# Autodesk Inventor assembly: Shooter Assembly
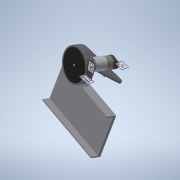
[picture p0: Inventor's stored thumbnail of the model, 180x180]
Saved by Autodesk Inventor 2021 (Build 250183000, 183)
## iProperties
Created: 2020-10-17
Part Number: Shooter Assembly
Document SubType Name: Assembly
Designer: Delta
Author: Delta
## Documents named in this file (12)
- D:\robotics\CAD\2020-21-CAD\Shooter\Shooter Assembly.iam
- D:\robotics\CAD\2020-21-CAD\Shooter\Guide.ipt
- D:\robotics\CAD\2020-21-CAD\Shooter\Axle Rotate.ipt
- D:\robotics\CAD\2020-21-CAD\Shooter\Triangle axle slide connector.ipt
- D:\robotics\CAD\2020-21-CAD\Shooter\Tetrex 2pc motor mount.ipt
- D:\robotics\CAD\2020-21-CAD\Shooter\motor-3102NeveRest20 (1).ipt
- D:\robotics\CAD\2020-21-CAD\Shooter\Flywheel_4inWheel8mmHub.ipt
- D:\robotics\CAD\2020-21-CAD\Shooter\Tetrix bracket - single servo.ipt
- D:\robotics\CAD\COTSParts\Rev\REV-41-1097SmartServo.ipt
- D:\robotics\CAD\2020-21-CAD\Shooter\Triangle connector.ipt
- D:\robotics\CAD\2020-21-CAD\Shooter\U bracket.ipt
- D:\robotics\CAD\2020-21-CAD\Shooter\Triangle connector 2.ipt
## Components (14 placed, 11 different names)
1. Guide:1 — Mate:14, Mate:15, Angle:1, Angle:2, Mate:37, Mate:38, Mate:39, Mate:40
2. Axle Rotate:1 — Mate:9, Mate:13, Mate:40
3. Axle Rotate:2 — Mate:8, Mate:12, Mate:37, Mate:38, Mate:39
4. Triangle axle slide connector:1 — Mate:8, Flush:2, Mate:12, Angle:3, Mate:34, Flush:5, Mate:35, Flush:7
5. Triangle axle slide connector:2 — Mate:9, Flush:2, Mate:13, Mate:24, Flush:3, Mate:30, Mate:31
6. Tetrex 2pc motor mount:1 — Mate:14, Mate:15, Angle:1, Mate:16, Mate:17
7. motor-3102NeveRest20 (1):1 — Mate:16, Mate:17, Mate:18, Mate:19, Angle:2
8. Flywheel_4inWheel8mmHub:1 — Mate:18, Mate:19
9. Tetrix bracket - single servo:1 — Mate:25, Mate:26, Mate:27, Angle:3, Mate:32, Flush:4
10. REV-41-1097SmartServo:1 — Mate:25, Mate:26, Mate:27, Mate:30
11. Triangle connector:1 — Mate:24, Flush:3, Mate:33, Flush:6
12. U bracket:1 — Mate:31, Mate:32, Flush:4, Mate:33
13. Triangle connector:2 — Mate:34, Flush:5, Flush:6, Mate:36
14. Triangle connector 2:1 — Mate:35, Flush:7, Mate:36
## Relationships (34: Mate 25, Flush 6, Angle 3)
- Mate:8: Axle Rotate:2 ↔ Triangle axle slide connector:1
- Mate:9: Axle Rotate:1 ↔ Triangle axle slide connector:2
- Flush:2: Triangle axle slide connector:1 ↔ Triangle axle slide connector:2
- Mate:12: Axle Rotate:2 ↔ Triangle axle slide connector:1
- Mate:13: Axle Rotate:1 ↔ Triangle axle slide connector:2
- Mate:14: Guide:1 ↔ Tetrex 2pc motor mount:1
- Mate:15: Guide:1 ↔ Tetrex 2pc motor mount:1
- Angle:1 (0 deg): Guide:1 ↔ Tetrex 2pc motor mount:1
- Mate:16: Tetrex 2pc motor mount:1 ↔ motor-3102NeveRest20 (1):1
- Mate:17: Tetrex 2pc motor mount:1 ↔ motor-3102NeveRest20 (1):1
- Mate:18: motor-3102NeveRest20 (1):1 ↔ Flywheel_4inWheel8mmHub:1
- Mate:19: motor-3102NeveRest20 (1):1 ↔ Flywheel_4inWheel8mmHub:1
- Angle:2 (0 deg): Guide:1 ↔ motor-3102NeveRest20 (1):1
- Mate:24: Triangle axle slide connector:2 ↔ Triangle connector:1
- Flush:3: Triangle axle slide connector:2 ↔ Triangle connector:1
- Mate:25: Tetrix bracket - single servo:1 ↔ REV-41-1097SmartServo:1
- Mate:26 (5.08 mm): Tetrix bracket - single servo:1 ↔ REV-41-1097SmartServo:1
- Mate:27 (-3.81 mm): Tetrix bracket - single servo:1 ↔ REV-41-1097SmartServo:1
- Mate:30: Triangle axle slide connector:2 ↔ REV-41-1097SmartServo:1
- Angle:3 (0 deg): Triangle axle slide connector:1 ↔ Tetrix bracket - single servo:1
- Mate:31: Triangle axle slide connector:2 ↔ U bracket:1
- Mate:32: Tetrix bracket - single servo:1 ↔ U bracket:1
- Flush:4 (25.4 mm): Tetrix bracket - single servo:1 ↔ U bracket:1
- Mate:33 (50.8 mm): Triangle connector:1 ↔ U bracket:1
- Mate:34: Triangle axle slide connector:1 ↔ Triangle connector:2
- Flush:5: Triangle axle slide connector:1 ↔ Triangle connector:2
- Flush:6: Triangle connector:1 ↔ Triangle connector:2
- Mate:35: Triangle axle slide connector:1 ↔ Triangle connector 2:1
- Flush:7: Triangle axle slide connector:1 ↔ Triangle connector 2:1
- Mate:36 (47.752 mm): Triangle connector:2 ↔ Triangle connector 2:1
- Mate:37: Guide:1 ↔ Axle Rotate:2
- Mate:38: Guide:1 ↔ Axle Rotate:2
- Mate:39: Guide:1 ↔ Axle Rotate:2
- Mate:40: Guide:1 ↔ Axle Rotate:1
